# Autodesk Inventor assembly: Frame
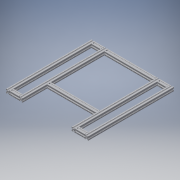
[picture p0: Inventor's stored thumbnail of the model, 180x180]
Saved by Autodesk Inventor 2017 (Build 210142000, 142)
## iProperties
Created: 2018-04-25
Part Number: Frame
Document SubType Name: Assembly
Designer: User
Author: User
## Documents named in this file (4)
- C:\Robotics\CAD\2018-19_CAD\Offseason\Frame.iam
- C:\Robotics\CAD\COTSParts\Bosch Extrusion\Bosch 20x20 17.5 in.ipt
- C:\Robotics\CAD\COTSParts\Bosch Extrusion\Bosch 20x20 1.875in.ipt
- C:\Robotics\CAD\COTSParts\Bosch Extrusion\Bosch 20x20 10in.ipt
## Components (10 placed, 3 different names)
1. Bosch 20x20 17.5 in:1 — Flush:2, Flush:3, Mate:5, Flush:9, Mate:7, Flush:12, Mate:9, Flush:18, Flush:19, Mate:10, Flush:21
2. Bosch 20x20 17.5 in:2 — Flush:1, Flush:2, Mate:6, Flush:10, Mate:8, Flush:11
3. Bosch 20x20 17.5 in:3 — Flush:3, Flush:4, Mate:2, Flush:8, Mate:4, Flush:17, Mate:11, Flush:20, Mate:12
4. Bosch 20x20 17.5 in:4 — Flush:4, Flush:5, Flush:6, Flush:7, Mate:1, Mate:3
5. Bosch 20x20 1.875in:1 — Flush:1, Mate:3, Mate:4, Flush:17
6. Bosch 20x20 1.875in:2 — Mate:7, Mate:8, Flush:11, Flush:12
7. Bosch 20x20 1.875in:3 — Flush:6, Mate:5, Mate:6, Flush:9, Flush:10
8. Bosch 20x20 1.875in:4 — Flush:5, Flush:7, Mate:1, Mate:2, Flush:8
9. Bosch 20x20 10in:1 — Flush:19, Mate:10, Mate:12, Flush:21
10. Bosch 20x20 10in:2 — Mate:9, Flush:18, Mate:11, Flush:20
## Relationships (29: Flush 17, Mate 12)
- Flush:1: Bosch 20x20 17.5 in:2 ↔ Bosch 20x20 1.875in:1
- Flush:2: Bosch 20x20 17.5 in:1 ↔ Bosch 20x20 17.5 in:2
- Flush:3: Bosch 20x20 17.5 in:1 ↔ Bosch 20x20 17.5 in:3
- Flush:4: Bosch 20x20 17.5 in:3 ↔ Bosch 20x20 17.5 in:4
- Flush:5: Bosch 20x20 17.5 in:4 ↔ Bosch 20x20 1.875in:4
- Flush:6: Bosch 20x20 17.5 in:4 ↔ Bosch 20x20 1.875in:3
- Flush:7: Bosch 20x20 17.5 in:4 ↔ Bosch 20x20 1.875in:4
- Mate:1: Bosch 20x20 17.5 in:4 ↔ Bosch 20x20 1.875in:4
- Mate:2: Bosch 20x20 17.5 in:3 ↔ Bosch 20x20 1.875in:4
- Flush:8: Bosch 20x20 17.5 in:3 ↔ Bosch 20x20 1.875in:4
- Mate:3: Bosch 20x20 17.5 in:4 ↔ Bosch 20x20 1.875in:1
- Mate:4: Bosch 20x20 17.5 in:3 ↔ Bosch 20x20 1.875in:1
- Mate:5: Bosch 20x20 17.5 in:1 ↔ Bosch 20x20 1.875in:3
- Mate:6: Bosch 20x20 17.5 in:2 ↔ Bosch 20x20 1.875in:3
- Flush:9: Bosch 20x20 17.5 in:1 ↔ Bosch 20x20 1.875in:3
- Flush:10: Bosch 20x20 17.5 in:2 ↔ Bosch 20x20 1.875in:3
- Mate:7: Bosch 20x20 17.5 in:1 ↔ Bosch 20x20 1.875in:2
- Mate:8: Bosch 20x20 17.5 in:2 ↔ Bosch 20x20 1.875in:2
- Flush:11: Bosch 20x20 17.5 in:2 ↔ Bosch 20x20 1.875in:2
- Flush:12: Bosch 20x20 17.5 in:1 ↔ Bosch 20x20 1.875in:2
- Flush:17: Bosch 20x20 17.5 in:3 ↔ Bosch 20x20 1.875in:1
- Mate:9: Bosch 20x20 17.5 in:1 ↔ Bosch 20x20 10in:2
- Flush:18: Bosch 20x20 17.5 in:1 ↔ Bosch 20x20 10in:2
- Flush:19: Bosch 20x20 17.5 in:1 ↔ Bosch 20x20 10in:1
- Mate:10: Bosch 20x20 17.5 in:1 ↔ Bosch 20x20 10in:1
- Mate:11: Bosch 20x20 17.5 in:3 ↔ Bosch 20x20 10in:2
- Flush:20: Bosch 20x20 17.5 in:3 ↔ Bosch 20x20 10in:2
- Mate:12: Bosch 20x20 17.5 in:3 ↔ Bosch 20x20 10in:1
- Flush:21 (127 mm): Bosch 20x20 17.5 in:1 ↔ Bosch 20x20 10in:1
